# Autodesk Inventor assembly: 4.1h_JulianR_Assemblypart5
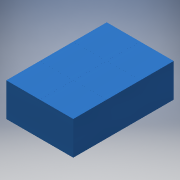
[picture p0: Inventor's stored thumbnail of the model, 180x180]
Saved by Autodesk Inventor 2016 (Build 200138000, 138)
## iProperties
Created: 2017-03-02
Part Number: 4.1h_JulianR_Assemblypart5
Document SubType Name: Assembly
Designer: fhs-mgr
Author: fhs-mgr
## Documents named in this file (2)
- H:\IED 5th Inventor\4.1h_JulianR_Assemblypart5.iam
- H:\IED 5th Inventor\WoodenBlock.ipt
## Components (6 placed, 1 different names)
1. WoodenBlock:1 — Mate:5, Mate:6, Mate:14
2. WoodenBlock:5 — Mate:5, Mate:6, Mate:7, Mate:8, Mate:11
3. WoodenBlock:6 — Mate:7, Mate:8, Mate:9, Mate:10
4. WoodenBlock:7 — Mate:13, Mate:14
5. WoodenBlock:8 — Mate:11, Mate:12, Mate:13
6. WoodenBlock:9 — Mate:9, Mate:10, Mate:12
## Relationships (10: Mate 10)
- Mate:5: WoodenBlock:1 ↔ WoodenBlock:5
- Mate:6: WoodenBlock:1 ↔ WoodenBlock:5
- Mate:7: WoodenBlock:5 ↔ WoodenBlock:6
- Mate:8: WoodenBlock:5 ↔ WoodenBlock:6
- Mate:9: WoodenBlock:6 ↔ WoodenBlock:9
- Mate:10: WoodenBlock:6 ↔ WoodenBlock:9
- Mate:11: WoodenBlock:5 ↔ WoodenBlock:8
- Mate:12: WoodenBlock:8 ↔ WoodenBlock:9
- Mate:13: WoodenBlock:7 ↔ WoodenBlock:8
- Mate:14: WoodenBlock:1 ↔ WoodenBlock:7
